# Autodesk Inventor assembly: Assembly_center_suspension
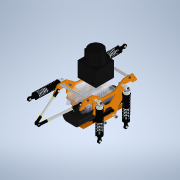
[picture p0: Inventor's stored thumbnail of the model, 180x180]
Saved by Autodesk Inventor 2020 (Build 240168000, 168)
## iProperties
Created: 2019-10-08
Part Number: Assembly_center_suspension
Document SubType Name: Assembly
Designer: maste
Author: maste
## Documents named in this file (21)
- C:\Users\maste\Documents\GitHub\autobot\robot_model\Assembly_center_suspension.iam
- C:\Users\maste\Documents\GitHub\autobot\robot_model\Assembly_center_unit.iam
- C:\Users\maste\Documents\GitHub\autobot\robot_model\RCT-H015_Tuerca_Conica.ipt
- C:\Users\maste\Documents\GitHub\autobot\robot_model\Ensamble_Amortiguador.iam
- C:\Users\maste\Documents\GitHub\autobot\robot_model\Assembly_center_suspension\Design Accelerator\cent_susp_BC001.iam
- C:\Users\maste\Documents\GitHub\autobot\robot_model\Assembly_center_suspension\Design Accelerator\cent_susp_BC002.iam
- C:\Users\maste\Documents\GitHub\autobot\robot_model\Assembly_center_suspension\Design Accelerator\cent_susp_BC003.iam
- C:\Users\maste\Documents\GitHub\autobot\robot_model\Assembly_center_suspension\Design Accelerator\cent_susp_BC004.iam
- C:\Users\maste\Documents\GitHub\autobot\robot_model\RCT-H022_washer_25_55_05.ipt
- C:\Users\maste\Documents\GitHub\autobot\robot_model\RCT-H017_lower_linkage_ball_stud.ipt
- C:\Users\maste\Documents\GitHub\autobot\robot_model\H205_lower_linkage_washer.ipt
- C:\Users\maste\Documents\GitHub\autobot\robot_model\Assembly_center_suspension\Design Accelerator\lower_linkage_ball_BC001.iam
- C:\Users\maste\Documents\GitHub\autobot\robot_model\Assembly_center_suspension\Design Accelerator\lower_linkage_ball_BC002.iam
- C:\Users\maste\Documents\GitHub\autobot\robot_model\Assembly_center_suspension\Design Accelerator\lower_linkage_ball_BC003.iam
- C:\Users\maste\Documents\GitHub\autobot\robot_model\Assembly_center_suspension\Design Accelerator\lower_linkage_ball_BC004.iam
- C:\Users\maste\Documents\GitHub\autobot\robot_model\foam_battery_base.ipt
- C:\Users\maste\Documents\GitHub\autobot\robot_model\HX-2000MHT.ipt
- C:\Users\maste\Documents\GitHub\autobot\robot_model\case_roboclaw_assembly.iam
- C:\Users\maste\Documents\GitHub\autobot\robot_model\Hokuyo Telemeter.ipt
- C:\Users\maste\Documents\GitHub\autobot\robot_model\H016 (2).ipt
- C:\Users\maste\Documents\GitHub\autobot\robot_model\Ensamblaje_eslabón.iam
## Components (37 placed, 13 different names)
1. Assembly_center_unit:1 [sub-assembly] — Mate:1, Mate:2, Mate:3, Mate:4, Mate:5, Mate:6, Mate:7, Mate:8, Mate:25, Mate:26, Mate:27, Mate:28, Mate:29, Mate:30, Mate:31, Mate:32, Mate:57, Mate:58, Flush:1, Flush:2, Mate:60, Mate:61, Mate:62, Mate:63
2. RCT-H015_Tuerca_Conica:1 — Mate:1, Mate:2, Mate:9, Mate:10
3. RCT-H015_Tuerca_Conica:2 — Mate:3, Mate:4, Mate:13, Mate:14
4. RCT-H015_Tuerca_Conica:3 — Mate:5, Mate:6, Mate:15, Mate:16
5. RCT-H015_Tuerca_Conica:4 — Mate:7, Mate:8, Mate:11, Mate:12
6. Ensamble_Amortiguador:1 [sub-assembly] — Mate:9, Mate:10, Mate:19, Mate:20
7. Ensamble_Amortiguador:2 [sub-assembly] — Mate:13, Mate:14, Mate:17, Mate:18
8. Ensamble_Amortiguador:3 [sub-assembly] — Mate:15, Mate:16, Mate:21, Mate:22
9. Ensamble_Amortiguador:4 [sub-assembly] — Mate:11, Mate:12, Mate:23, Mate:24
10. Bolted Connection:1 [sub-assembly] — Mate:17, Mate:18
11. Bolted Connection:2 [sub-assembly] — Mate:19, Mate:20
12. Bolted Connection:3 [sub-assembly] — Mate:21, Mate:22
13. Bolted Connection:4 [sub-assembly] — Mate:23, Mate:24
14. RCT-H022_washer_25_55_05:1 — Mate:25, Mate:29, Mate:33, Mate:35
15. RCT-H022_washer_25_55_05:2 — Mate:26, Mate:30, Mate:34, Mate:36
16. RCT-H022_washer_25_55_05:3 — Mate:28, Mate:31, Mate:38, Mate:40
17. RCT-H022_washer_25_55_05:4 — Mate:27, Mate:32, Mate:37, Mate:39
18. RCT-H017_lower_linkage_ball_stud:1 — Mate:33, Mate:35, Mate:41, Mate:44
19. RCT-H017_lower_linkage_ball_stud:2 — Mate:34, Mate:36, Mate:42, Mate:43
20. RCT-H017_lower_linkage_ball_stud:3 — Mate:37, Mate:39, Mate:46, Mate:48
21. RCT-H017_lower_linkage_ball_stud:4 — Mate:38, Mate:40, Mate:45, Mate:47
22. H205_lower_linkage_washer:1 — Mate:41, Mate:44, Mate:51, Mate:52
23. H205_lower_linkage_washer:2 — Mate:42, Mate:43, Mate:49, Mate:50
24. H205_lower_linkage_washer:3 — Mate:45, Mate:47, Mate:55, Mate:56
25. H205_lower_linkage_washer:4 — Mate:46, Mate:48, Mate:53, Mate:54
26. Bolted Connection:5 [sub-assembly] — Mate:49, Mate:50
27. Bolted Connection:6 [sub-assembly] — Mate:51, Mate:52
28. Bolted Connection:7 [sub-assembly] — Mate:53, Mate:54
29. Bolted Connection:8 [sub-assembly] — Mate:55, Mate:56
30. foam_battery_base:1 — Mate:57, Mate:58, Flush:1, Mate:59
31. HX-2000MHT:1 — Mate:59, Flush:2
32. case_roboclaw_assembly:1 [sub-assembly]
33. Hokuyo Telemeter:1
34. H016 (2):1 — Mate:60, Mate:61, Ball:1, Angle:1
35. Ensamblaje_eslabón:1 [sub-assembly] — Ball:1, Angle:1
36. H016 (2):2 — Mate:62, Mate:63, Ball:2, Angle:2
37. Ensamblaje_eslabón:2 [sub-assembly] — Ball:2, Angle:2
## Relationships (69: Mate 63, Flush 2, BallJoint 2, Angle 2)
- Mate:1: Assembly_center_unit:1 ↔ RCT-H015_Tuerca_Conica:1
- Mate:2: Assembly_center_unit:1 ↔ RCT-H015_Tuerca_Conica:1
- Mate:3: Assembly_center_unit:1 ↔ RCT-H015_Tuerca_Conica:2
- Mate:4: Assembly_center_unit:1 ↔ RCT-H015_Tuerca_Conica:2
- Mate:5: Assembly_center_unit:1 ↔ RCT-H015_Tuerca_Conica:3
- Mate:6: Assembly_center_unit:1 ↔ RCT-H015_Tuerca_Conica:3
- Mate:7: Assembly_center_unit:1 ↔ RCT-H015_Tuerca_Conica:4
- Mate:8: Assembly_center_unit:1 ↔ RCT-H015_Tuerca_Conica:4
- Mate:9: RCT-H015_Tuerca_Conica:1 ↔ Ensamble_Amortiguador:1
- Mate:10: RCT-H015_Tuerca_Conica:1 ↔ Ensamble_Amortiguador:1
- Mate:11: RCT-H015_Tuerca_Conica:4 ↔ Ensamble_Amortiguador:4
- Mate:12: RCT-H015_Tuerca_Conica:4 ↔ Ensamble_Amortiguador:4
- Mate:13: RCT-H015_Tuerca_Conica:2 ↔ Ensamble_Amortiguador:2
- Mate:14: RCT-H015_Tuerca_Conica:2 ↔ Ensamble_Amortiguador:2
- Mate:15: RCT-H015_Tuerca_Conica:3 ↔ Ensamble_Amortiguador:3
- Mate:16: RCT-H015_Tuerca_Conica:3 ↔ Ensamble_Amortiguador:3
- Mate:17: Ensamble_Amortiguador:2 ↔ Bolted Connection:1
- Mate:18: Ensamble_Amortiguador:2 ↔ Bolted Connection:1
- Mate:19: Ensamble_Amortiguador:1 ↔ Bolted Connection:2
- Mate:20: Ensamble_Amortiguador:1 ↔ Bolted Connection:2
- Mate:21: Ensamble_Amortiguador:3 ↔ Bolted Connection:3
- Mate:22: Ensamble_Amortiguador:3 ↔ Bolted Connection:3
- Mate:23: Ensamble_Amortiguador:4 ↔ Bolted Connection:4
- Mate:24: Ensamble_Amortiguador:4 ↔ Bolted Connection:4
- Mate:25: Assembly_center_unit:1 ↔ RCT-H022_washer_25_55_05:1
- Mate:26: Assembly_center_unit:1 ↔ RCT-H022_washer_25_55_05:2
- Mate:27: Assembly_center_unit:1 ↔ RCT-H022_washer_25_55_05:4
- Mate:28: Assembly_center_unit:1 ↔ RCT-H022_washer_25_55_05:3
- Mate:29: Assembly_center_unit:1 ↔ RCT-H022_washer_25_55_05:1
- Mate:30: Assembly_center_unit:1 ↔ RCT-H022_washer_25_55_05:2
- Mate:31: Assembly_center_unit:1 ↔ RCT-H022_washer_25_55_05:3
- Mate:32: Assembly_center_unit:1 ↔ RCT-H022_washer_25_55_05:4
- Mate:33: RCT-H022_washer_25_55_05:1 ↔ RCT-H017_lower_linkage_ball_stud:1
- Mate:34: RCT-H022_washer_25_55_05:2 ↔ RCT-H017_lower_linkage_ball_stud:2
- Mate:35: RCT-H022_washer_25_55_05:1 ↔ RCT-H017_lower_linkage_ball_stud:1
- Mate:36: RCT-H022_washer_25_55_05:2 ↔ RCT-H017_lower_linkage_ball_stud:2
- Mate:37: RCT-H022_washer_25_55_05:4 ↔ RCT-H017_lower_linkage_ball_stud:3
- Mate:38: RCT-H022_washer_25_55_05:3 ↔ RCT-H017_lower_linkage_ball_stud:4
- Mate:39: RCT-H022_washer_25_55_05:4 ↔ RCT-H017_lower_linkage_ball_stud:3
- Mate:40: RCT-H022_washer_25_55_05:3 ↔ RCT-H017_lower_linkage_ball_stud:4
- Mate:41: RCT-H017_lower_linkage_ball_stud:1 ↔ H205_lower_linkage_washer:1
- Mate:42: RCT-H017_lower_linkage_ball_stud:2 ↔ H205_lower_linkage_washer:2
- Mate:43: RCT-H017_lower_linkage_ball_stud:2 ↔ H205_lower_linkage_washer:2
- Mate:44: RCT-H017_lower_linkage_ball_stud:1 ↔ H205_lower_linkage_washer:1
- Mate:45: RCT-H017_lower_linkage_ball_stud:4 ↔ H205_lower_linkage_washer:3
- Mate:46: RCT-H017_lower_linkage_ball_stud:3 ↔ H205_lower_linkage_washer:4
- Mate:47: RCT-H017_lower_linkage_ball_stud:4 ↔ H205_lower_linkage_washer:3
- Mate:48: RCT-H017_lower_linkage_ball_stud:3 ↔ H205_lower_linkage_washer:4
- Mate:49: H205_lower_linkage_washer:2 ↔ Bolted Connection:5
- Mate:50: H205_lower_linkage_washer:2 ↔ Bolted Connection:5
- Mate:51: H205_lower_linkage_washer:1 ↔ Bolted Connection:6
- Mate:52: H205_lower_linkage_washer:1 ↔ Bolted Connection:6
- Mate:53: H205_lower_linkage_washer:4 ↔ Bolted Connection:7
- Mate:54: H205_lower_linkage_washer:4 ↔ Bolted Connection:7
- Mate:55: H205_lower_linkage_washer:3 ↔ Bolted Connection:8
- Mate:56: H205_lower_linkage_washer:3 ↔ Bolted Connection:8
- Mate:57: Assembly_center_unit:1 ↔ foam_battery_base:1
- Mate:58: Assembly_center_unit:1 ↔ foam_battery_base:1
- Flush:1: Assembly_center_unit:1 ↔ foam_battery_base:1
- Mate:59: foam_battery_base:1 ↔ HX-2000MHT:1
- Flush:2 (-10 mm): Assembly_center_unit:1 ↔ HX-2000MHT:1
- Mate:60: Assembly_center_unit:1 ↔ H016 (2):1
- Mate:61: Assembly_center_unit:1 ↔ H016 (2):1
- Ball:1: H016 (2):1 ↔ Ensamblaje_eslabón:1
- Angle:1 (0 deg): H016 (2):1 ↔ Ensamblaje_eslabón:1
- Mate:62: Assembly_center_unit:1 ↔ H016 (2):2
- Mate:63: Assembly_center_unit:1 ↔ H016 (2):2
- Ball:2: H016 (2):2 ↔ Ensamblaje_eslabón:2
- Angle:2 (0 deg): H016 (2):2 ↔ Ensamblaje_eslabón:2
